# Autodesk Inventor assembly: EstanteColgado
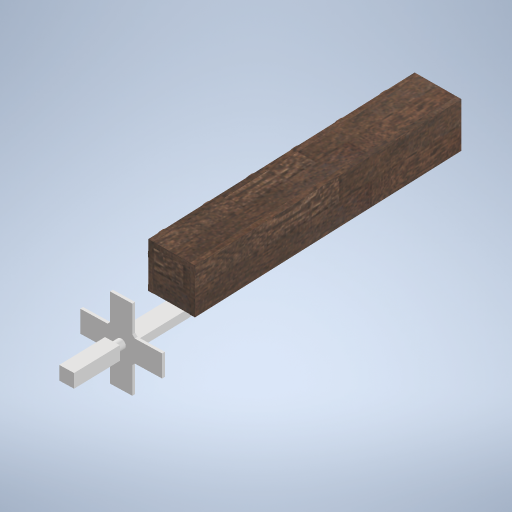
[picture p0: Inventor's stored thumbnail of the model, 512x512]
Saved by Autodesk Inventor 2023 (Build 270158000, 158)
## iProperties
Created: 2023-05-30
Part Number: EstanteColgado
Document SubType Name: Assembly
Designer: WIN10
Author: WIN10
## Documents named in this file (3)
- C:\Users\WIN10\DisenoDeProduccion\ModelosCeldaRobotica\EstanteColgado.iam
- G:\Unidades compartidas\Amiguitos por siempre\APM 2023-1\Piezas\RepisaLego.iam
- C:\Users\WIN10\DisenoDeProduccion\ModelosCeldaRobotica\Gancho.ipt
## Components (2 placed, 2 different names)
1. RepisaLego:1 [sub-assembly] — Coincidencia:1
2. Gancho:1 — Coincidencia:1
## Relationships (1: Mate 1)
- Coincidencia:1 [Mate]: RepisaLego:1 ↔ Gancho:1
